# Autodesk Inventor assembly: Montagem
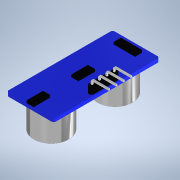
[picture p0: Inventor's stored thumbnail of the model, 180x180]
Saved by Autodesk Inventor 2021 (Build 250183000, 183)
## iProperties
Created: 2021-06-10
Part Number: Montagem
Document SubType Name: Assembly
Designer: rubia
Author: rubia
## Documents named in this file (4)
- C:\Users\rubia\OneDrive\Documentos\201910663_Semestral\Montagem.iam
- C:\Users\rubia\OneDrive\Documentos\201910663_Semestral\Caixa.ipt
- C:\Users\rubia\OneDrive\Documentos\201910663_Semestral\Conector.ipt
- C:\Users\rubia\OneDrive\Documentos\201910663_Semestral\Placa.ipt
## Components (4 placed, 3 different names)
1. Caixa:1 — Coincidente:2, Alinhado:3, Coincidente:3
2. Conector:1 — Coincidente:4, Coincidente:5, Coincidente:6
3. Placa:1 — Coincidente:1, Coincidente:2, Alinhado:1, Alinhado:2, Alinhado:3, Coincidente:3, Coincidente:4, Coincidente:5, Coincidente:6
4. Caixa:2 — Coincidente:1, Alinhado:1, Alinhado:2
## Relationships (9: Mate 6, Flush 3)
- Coincidente:1 [Mate]: Placa:1 ↔ Caixa:2
- Coincidente:2 [Mate]: Caixa:1 ↔ Placa:1
- Alinhado:1 [Flush] (9 mm): Placa:1 ↔ Caixa:2
- Alinhado:2 [Flush] (10 mm): Placa:1 ↔ Caixa:2
- Alinhado:3 [Flush] (10 mm): Caixa:1 ↔ Placa:1
- Coincidente:3 [Mate] (-9 mm): Caixa:1 ↔ Placa:1
- Coincidente:4 [Mate]: Conector:1 ↔ Placa:1
- Coincidente:5 [Mate] (-0.5 mm): Conector:1 ↔ Placa:1
- Coincidente:6 [Mate] (-17.5 mm): Conector:1 ↔ Placa:1
